# Autodesk Inventor assembly: LWLF42...BCS1710(100,0,0)I
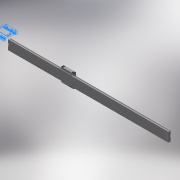
[picture p0: Inventor's stored thumbnail of the model, 180x180]
Saved by Autodesk Inventor 2016 (Build 200138000, 138)
## iProperties
Category: PARTsolutions
Company: IKO
Created: 2015-04-20
Part Number: LWLF42...BCS1710(100,0,0)I
Catalog Web Link: www.cadenas.de
Description: Interchangeable, Assembled set-LWLF42...BCS
Vendor: IKO
Document SubType Name: Assembly
Designer: PARTuser1
Manufacturer: IKO
PSOL_IDENT_0: {$CADENAS_DATA\23d-libs\iko\linear_way_series\linear_way_l_series\lwlf\lwlf42_bcs\lwlf42bcs_i_asmtab
PSOL_IDENT_1: .prj},240 {VTYP=3D},{STYP=ASSTAB},{NB=LWLF42...BCS1710(100,0,0)I},{LINA=LWLF42C1R710BCSS1},{NN=Inter
PSOL_IDENT_2: changeable, Assembled set},{DATE=11.12.2014 01:21:41},{GEOMDATE=16.10.2008},{VERSION=},{LINEID=80},{
PSOL_IDENT_3: LINESUBID=-1},{WBVAR=NS,REF,ES,CP,US,L,P1,P2,P3}  {NB=LWLF42...BCS1710(100,0,0)I},{LINA=LWLF42C1R710
PSOL_IDENT_4: BCSS1},{KT=DUMMY},{MN=LWLF42},{MNX=LWLF42...BCS},{NS=1},{REF=},{ES=},{CP=},{US=},{L=710.00},{SP=},{P
PSOL_IDENT_5: 1=100.000},{P2=0.000},{P3=0.000},{H=16.0},{H1=4.0},{NSL=9.0},{W2=60},{W3=45},{W4=7.5},{L1=54.80},{L2=
PSOL_IDENT_6: 20.0},{L3=39.0},{L4=60.00},{M1=4.00},{DPTH=4.50},{H3=3.2},{W=42},{H4=10.0},{D3=4.5},{D4=8.0},{HM=4.5
PSOL_IDENT_7: 0},{LEND=1560.000},{LMIN=60},{PSM1=27.4},{PSM2=0},{PSM3=0},{PS1=682.6},{PS2=0},{PS3=0},{P2X=0},{P3X=
PSOL_IDENT_8: 0},{BJ=},{A=5.000},{C=2.000},{ES1='', 'No', 'N', 'Yes'},{CP1='', 'No', 'Q', 'Yes'},{SP1='', 'No', 'S'
PSOL_IDENT_9: , 'Yes'},{LXSP=0},{E1=15},{E2=15},{EK=30},{ED=20},{ED1=0},{EMIND=6.5},{LX=680},{LY=1520},{LZ=1560},{
PSOL_IDENT_10: LS=1520.000},{LV=2230},{LMINS=72},{LMAX=1600.000},{NMAX=1.000},{F=40},{ENOM=20.000},{EMIN=6.500},{EM
PSOL_IDENT_11: INJ=6.500},{EMAXJ=26.500},{N=1},{P=18},{PV=110},{L1D=1075},{L4D=1155},{H4D=1.000},{H1D=1.000},{P1D=5
PSOL_IDENT_12: 3},{P4D=57},{PS=38},{P1D1=55},{N1=1},{NX=1},{US1='', 'No', 'U', 'Yes'},{KC=},{PSM1X=27.4},{Q=4.40},{
PSOL_IDENT_13: QS=0.60},{LMINX1=60.00},{LMINQ1=70.00},{LMINX2=120.00},{LMINQ2=140.00},{LMINX3=180.00},{LMINQ3=210.0
PSOL_IDENT_14: 0},{L4L1=5.2},{L1X=54.8},{USX=2.00},{PPATH=lwlf_asmtpl.prj}
SUPPLIER: IKO
ARTICLENO: LWLF42...BCS1710(100,0,0)I
BOMINFO: LWLF42C1R710BCSS1
CREATOR: CADENAS GmbH
Title: LWLF42C1R710BCSS1
Author: Cadenas PARTsolutions
Comments: LWLF42...BCS
## Documents named in this file (3)
- C:\Users\ax\Documents\Inventor\components\IKO_LWLF42BCS171010000I\LWLF42___BCS1710_100_0_0_I.iam
- C:\Users\ax\Documents\Inventor\components\IKO_LWLF42BCS171010000I\LWLF42___BCSR710Track_Rail.ipt
- C:\Users\ax\Documents\Inventor\components\IKO_LWLF42BCS171010000I\LWLF42___BCSR_Slide_Unit.ipt
## Components (2 placed, 2 different names)
1. LWLF42___BCSR710Track_Rail:1 — Slider:1, Mate:1, Mate:2
2. LWLF42___BCSR_Slide_Unit:1 — Slider:1, Mate:1, Mate:2
## Relationships (3: Mate 2, TranslationJoint 1)
- Slider:1 [TranslationJoint] (1 mm): LWLF42___BCSR710Track_Rail:1 ↔ LWLF42___BCSR_Slide_Unit:1
- Mate:1 (0.4 mm): LWLF42___BCSR710Track_Rail:1 ↔ LWLF42___BCSR_Slide_Unit:1
- Mate:2 (0.4 mm): LWLF42___BCSR710Track_Rail:1 ↔ LWLF42___BCSR_Slide_Unit:1
